# Autodesk Inventor assembly: ehlers
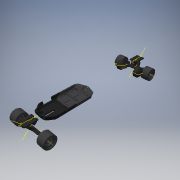
[picture p0: Inventor's stored thumbnail of the model, 180x180]
Saved by Autodesk Inventor 2016 (Build 200138000, 138)
## iProperties
Created: 2015-07-18
Part Number: ehlers
Document SubType Name: Assembly
Designer: brent
Author: brent
## Documents named in this file (6)
- D:\Users\brent\OneDrive\electric-longboard\brent\v2\ehlers.iam
- D:\Users\brent\OneDrive\electric-longboard\brent\v2\ehlers_enclosure.ipt
- D:\Users\brent\OneDrive\electric-longboard\brent\v2\50cal.iam
- D:\Users\brent\OneDrive\electric-longboard\brent\v2\pulley_cover2.ipt
- D:\Users\brent\OneDrive\electric-longboard\brent\v2\mount_alt.ipt
- D:\Users\brent\OneDrive\electric-longboard\dliu\Board\Wheel Blank Pro 83mm.ipt
## Components (11 placed, 5 different names)
1. ehlers_enclosure:1 — Mate:1, Mate:2, Mate:3, Mate:4, Mate:5, Mate:6
2. 50cal:1 [sub-assembly] — Mate:1, Mate:2, Mate:3, Mate:21, Mate:22
3. 50cal:2 [sub-assembly] — Mate:4, Mate:5, Mate:6, Mate:13, Mate:16, Mate:17, Mate:18, Mate:19, Mate:20
4. pulley_cover2:1 — Mate:11, Mate:12, Mate:15
5. mount_alt:1 — Mate:11, Mate:12, Mate:15, Mate:16, Mate:17, Flush:1
6. pulley_cover2:2 — Mate:7, Mate:8, Mate:9
7. mount_alt:2 — Mate:7, Mate:8, Mate:9, Mate:13, Mate:18, Flush:1
8. Wheel Blank Pro 83mm:1 — Mate:22
9. Wheel Blank Pro 83mm:2 — Mate:20
10. Wheel Blank Pro 83mm:3 — Mate:19
11. Wheel Blank Pro 83mm:4 — Mate:21
## Relationships (21: Mate 20, Flush 1)
- Mate:1: ehlers_enclosure:1 ↔ 50cal:1
- Mate:2: ehlers_enclosure:1 ↔ 50cal:1
- Mate:3: ehlers_enclosure:1 ↔ 50cal:1
- Mate:4: ehlers_enclosure:1 ↔ 50cal:2
- Mate:5: ehlers_enclosure:1 ↔ 50cal:2
- Mate:6: ehlers_enclosure:1 ↔ 50cal:2
- Mate:7: pulley_cover2:2 ↔ mount_alt:2
- Mate:8: pulley_cover2:2 ↔ mount_alt:2
- Mate:9: pulley_cover2:2 ↔ mount_alt:2
- Mate:11: pulley_cover2:1 ↔ mount_alt:1
- Mate:12: pulley_cover2:1 ↔ mount_alt:1
- Mate:13: 50cal:2 ↔ mount_alt:2
- Mate:15: pulley_cover2:1 ↔ mount_alt:1
- Mate:16: 50cal:2 ↔ mount_alt:1
- Mate:17: 50cal:2 ↔ mount_alt:1
- Mate:18: 50cal:2 ↔ mount_alt:2
- Flush:1: mount_alt:1 ↔ mount_alt:2
- Mate:19: 50cal:2 ↔ Wheel Blank Pro 83mm:3
- Mate:20: 50cal:2 ↔ Wheel Blank Pro 83mm:2
- Mate:21: 50cal:1 ↔ Wheel Blank Pro 83mm:4
- Mate:22: 50cal:1 ↔ Wheel Blank Pro 83mm:1
